# Autodesk Inventor assembly: 9P 18T Sprocket, Circle_MIR
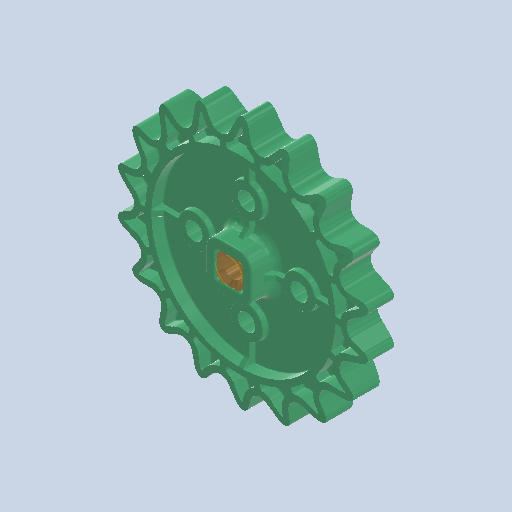
[picture p0: Inventor's stored thumbnail of the model, 512x512]
Saved by Autodesk Inventor 2024 (Build 280153000, 153)
## iProperties
Created: 2022-08-02
Part Number: 9P 18T Sprocket, Circle_MIR
Document SubType Name: Assembly
Designer: ismae
Author: ylu12
## Documents named in this file (3)
- C:\Users\ismae\Desktop\VEX\CAD 2023\VEX-CAD-Inventor\Motion\Sprockets\9P Sprocket\9P 18T Sprocket, Circle_MIR.iam
- C:\Users\ismae\Desktop\VEX\CAD 2023\VEX-CAD-Inventor\Motion\HS Shaft Adapter Circle_MIR.ipt
- C:\Users\ismae\Desktop\VEX\CAD 2023\VEX-CAD-Inventor\Motion\Sprockets\Reference Files\9P 18T Sprocket, No Insert_MIR.ipt
## Components (2 placed, 2 different names)
1. HS Shaft Adapter Circle_MIR:1 — Nivelación:1, Coincidencia:2, Coincidencia:1
2. 9P 18T Sprocket, No Insert_MIR:1 — Coincidencia:10, Coincidencia:9, Nivelación:5
## Relationships (6: Mate 4, Flush 2)
- Nivelación:1 [Flush] (-6.35 mm): HS Shaft Adapter Circle_MIR:1
- Coincidencia:2 [Mate]: HS Shaft Adapter Circle_MIR:1
- Coincidencia:1 [Mate]: HS Shaft Adapter Circle_MIR:1
- Coincidencia:10 [Mate]: 9P 18T Sprocket, No Insert_MIR:1
- Coincidencia:9 [Mate]: 9P 18T Sprocket, No Insert_MIR:1
- Nivelación:5 [Flush]: 9P 18T Sprocket, No Insert_MIR:1
